# Autodesk Inventor assembly: Ensamblaje
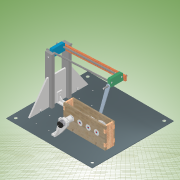
[picture p0: Inventor's stored thumbnail of the model, 180x180]
Saved by Autodesk Inventor 2022 (Build 260153000, 153)
## iProperties
Created: 2022-02-04
Part Number: Ensamblaje
Document SubType Name: Assembly
Designer: Marco
Author: Marco
## Documents named in this file (24)
- C:\Users\steff\Desktop\9noSemestre\Diseño\MiniProyecto\Ensamblaje.iam
- C:\Users\steff\Desktop\9noSemestre\Diseño\MiniProyecto\SoporteDerecha.ipt
- C:\Users\steff\Desktop\9noSemestre\Diseño\MiniProyecto\Varilla.ipt
- C:\Users\steff\Desktop\9noSemestre\Diseño\MiniProyecto\Riel_Lateral_MDF.ipt
- C:\Users\steff\Desktop\9noSemestre\Diseño\MiniProyecto\ColumnaSoporte.ipt
- C:\Users\steff\Desktop\9noSemestre\Diseño\MiniProyecto\SoporteIzquierda.ipt
- C:\Users\steff\Desktop\9noSemestre\Diseño\MiniProyecto\UnionColumnas.ipt
- C:\Users\steff\Desktop\9noSemestre\Diseño\MiniProyecto\SoporteMotor.ipt
- C:\Users\steff\Desktop\9noSemestre\Diseño\MiniProyecto\BaseProyecto.ipt
- C:\Users\steff\Desktop\9noSemestre\Diseño\MiniProyecto\CaraLateral.ipt
- C:\Users\steff\Desktop\9noSemestre\Diseño\MiniProyecto\Caja_CaraFrontal.ipt
- C:\Users\steff\Desktop\9noSemestre\Diseño\MiniProyecto\Rodamiento.ipt
- C:\Users\steff\Desktop\9noSemestre\Diseño\MiniProyecto\AcopleRod.ipt
- C:\Users\steff\Desktop\9noSemestre\Diseño\MiniProyecto\Eje.ipt
- C:\Users\steff\Desktop\9noSemestre\Diseño\MiniProyecto\Piñon1.ipt
- C:\Users\steff\Desktop\9noSemestre\Diseño\MiniProyecto\Archivos STL\EngranajesPegados.iam
- C:\Users\steff\Desktop\9noSemestre\Diseño\MiniProyecto\Engranaje1.ipt
- C:\Users\steff\Desktop\9noSemestre\Diseño\MiniProyecto\Transmision_Inf.ipt
- C:\Users\steff\Desktop\9noSemestre\Diseño\MiniProyecto\Transmision_Sup.ipt
- C:\Users\steff\Desktop\9noSemestre\Diseño\MiniProyecto\VarillaLateral.ipt
- C:\Users\steff\Desktop\9noSemestre\Diseño\MiniProyecto\AcopleMotor.ipt
- C:\Users\steff\Desktop\9noSemestre\Diseño\MiniProyecto\MotorDC.ipt
- C:\Users\steff\Desktop\9noSemestre\Diseño\MiniProyecto\SoporteMotorCierre.ipt
- C:\Users\steff\Desktop\9noSemestre\Diseño\MiniProyecto\Escuadra.ipt
## Components (44 placed, 23 different names)
1. BaseProyecto:1 — Coincidencia:1, Coincidencia:2, Coincidencia:3, Coincidencia:4, Coincidencia:5, Coincidencia:6, Coincidencia:13, Coincidencia:14, Coincidencia:15, Coincidencia:32, Coincidencia:33, Coincidencia:59
2. CaraLateral:1 — Coincidencia:1, Coincidencia:2, Coincidencia:3, Coincidencia:7, Coincidencia:8, Coincidencia:9, Coincidencia:11, Coincidencia:12, Coincidencia:34, Coincidencia:35, Coincidencia:36, Coincidencia:37, Coincidencia:38, Coincidencia:39, Coincidencia:40, Coincidencia:41
3. CaraLateral:2 — Coincidencia:4, Coincidencia:5, Coincidencia:6, Coincidencia:10, Coincidencia:42, Coincidencia:43, Coincidencia:44, Coincidencia:45, Coincidencia:46, Coincidencia:47
4. Caja_CaraFrontal:1 — Coincidencia:10, Coincidencia:11, Coincidencia:12
5. Caja_CaraFrontal:2 — Coincidencia:7, Coincidencia:8, Coincidencia:9
6. ColumnaSoporte:1 — Coincidencia:16, Coincidencia:17, De rotación:1, Coincidencia:20, Coincidencia:21, Coincidencia:51, Coincidencia:52
7. ColumnaSoporte:2 — Coincidencia:18, Coincidencia:19, Coincidencia:22, Coincidencia:23
8. UnionColumnas:1 — Coincidencia:13, Coincidencia:14, Coincidencia:15, Coincidencia:16, Coincidencia:17, Coincidencia:18, Coincidencia:19, Coincidencia:21, Coincidencia:22, Coincidencia:58, Coincidencia:60
9. SoporteIzquierda:1 — De rotación:1, De rotación:2, Coincidencia:20, Coincidencia:24, Coincidencia:25
10. Riel_Lateral_MDF:1 — De rotación:2, Coincidencia:23, Coincidencia:26, Coincidencia:27, Coincidencia:53
11. SoporteDerecha:1 — Coincidencia:26, Coincidencia:27, Coincidencia:28, Coincidencia:29, Coincidencia:30, Coincidencia:31, Coincidencia:49
12. Varilla:1 — Coincidencia:25, Coincidencia:29, Coincidencia:30
13. Varilla:2 — Coincidencia:24, Coincidencia:28, Coincidencia:31
14. SoporteMotor:1 — Coincidencia:32, Coincidencia:33, Coincidencia:54, Coincidencia:55, Coincidencia:56, Coincidencia:57
15. Rodamiento:1 — Coincidencia:34, Coincidencia:38, De rotación:3
16. Rodamiento:2 — Coincidencia:35, Coincidencia:39, De rotación:4
17. Rodamiento:3 — Coincidencia:37, Coincidencia:41, De rotación:6
18. Rodamiento:4 — Coincidencia:36, Coincidencia:40, De rotación:5
19. Rodamiento:5 — Coincidencia:46, Coincidencia:47, De rotación:9
20. Rodamiento:6 — Coincidencia:44, Coincidencia:45, De rotación:8
21. Rodamiento:8 — Coincidencia:42, Coincidencia:43, De rotación:7, De rotación:10
22. AcopleRod:1 — De rotación:6, Rígido:4
23. AcopleRod:2 — De rotación:4, Rígido:3
24. AcopleRod:3 — De rotación:5, Rígido:1
25. AcopleRod:4 — De rotación:3, Rígido:2
26. AcopleRod:5 — De rotación:7
27. AcopleRod:6 — De rotación:9
28. AcopleRod:7 — De rotación:8
29. Eje:4 — Rígido:1, Rígido:8
30. Eje:5 — Rígido:2, Rígido:5, Rígido:9
31. Eje:6 — Rígido:3, Rígido:6
32. Eje:7 — Rígido:4, Rígido:7
33. Piñon1:1 — Rígido:5
34. EngranajesPegados:1 [sub-assembly] — Rígido:8
35. EngranajesPegados:2 [sub-assembly] — Rígido:6
36. Engranaje1:1 — Rígido:7
37. Transmision_Inf:1 — De rotación:10, Coincidencia:48, De rotación:11
38. Transmision_Sup:1 — Coincidencia:48, De rotación:11, Coincidencia:49, Coincidencia:50
39. VarillaLateral:1 — Coincidencia:51, Coincidencia:52
40. VarillaLateral:2 — Coincidencia:50, Coincidencia:53
41. AcopleMotor:1 — Rígido:9
42. MotorDC:1 — Coincidencia:54, Coincidencia:55
43. SoporteMotorCierre:1 — Coincidencia:56, Coincidencia:57
44. Escuadra:1 — Coincidencia:58, Coincidencia:59, Coincidencia:60
## Relationships (80: Mate 60, RevoluteJoint 11, WeldJoint 9)
- Coincidencia:1 [Mate]: BaseProyecto:1 ↔ CaraLateral:1
- Coincidencia:2 [Mate]: BaseProyecto:1 ↔ CaraLateral:1
- Coincidencia:3 [Mate]: BaseProyecto:1 ↔ CaraLateral:1
- Coincidencia:4 [Mate]: BaseProyecto:1 ↔ CaraLateral:2
- Coincidencia:5 [Mate]: BaseProyecto:1 ↔ CaraLateral:2
- Coincidencia:6 [Mate]: BaseProyecto:1 ↔ CaraLateral:2
- Coincidencia:7 [Mate]: CaraLateral:1 ↔ Caja_CaraFrontal:2
- Coincidencia:8 [Mate]: CaraLateral:1 ↔ Caja_CaraFrontal:2
- Coincidencia:9 [Mate]: CaraLateral:1 ↔ Caja_CaraFrontal:2
- Coincidencia:10 [Mate]: CaraLateral:2 ↔ Caja_CaraFrontal:1
- Coincidencia:11 [Mate]: CaraLateral:1 ↔ Caja_CaraFrontal:1
- Coincidencia:12 [Mate]: CaraLateral:1 ↔ Caja_CaraFrontal:1
- Coincidencia:13 [Mate]: BaseProyecto:1 ↔ UnionColumnas:1
- Coincidencia:14 [Mate]: BaseProyecto:1 ↔ UnionColumnas:1
- Coincidencia:15 [Mate]: BaseProyecto:1 ↔ UnionColumnas:1
- Coincidencia:16 [Mate]: ColumnaSoporte:1 ↔ UnionColumnas:1
- Coincidencia:17 [Mate]: ColumnaSoporte:1 ↔ UnionColumnas:1
- Coincidencia:18 [Mate]: ColumnaSoporte:2 ↔ UnionColumnas:1
- Coincidencia:19 [Mate]: ColumnaSoporte:2 ↔ UnionColumnas:1
- De rotación:1 [RevoluteJoint]: ColumnaSoporte:1 ↔ SoporteIzquierda:1
- De rotación:2 [RevoluteJoint]: SoporteIzquierda:1 ↔ Riel_Lateral_MDF:1
- Coincidencia:20 [Mate]: ColumnaSoporte:1 ↔ SoporteIzquierda:1
- Coincidencia:21 [Mate]: ColumnaSoporte:1 ↔ UnionColumnas:1
- Coincidencia:22 [Mate]: ColumnaSoporte:2 ↔ UnionColumnas:1
- Coincidencia:23 [Mate]: ColumnaSoporte:2 ↔ Riel_Lateral_MDF:1
- Coincidencia:24 [Mate]: SoporteIzquierda:1 ↔ Varilla:2
- Coincidencia:25 [Mate]: SoporteIzquierda:1 ↔ Varilla:1
- Coincidencia:26 [Mate]: Riel_Lateral_MDF:1 ↔ SoporteDerecha:1
- Coincidencia:27 [Mate]: Riel_Lateral_MDF:1 ↔ SoporteDerecha:1
- Coincidencia:28 [Mate]: SoporteDerecha:1 ↔ Varilla:2
- Coincidencia:29 [Mate]: SoporteDerecha:1 ↔ Varilla:1
- Coincidencia:30 [Mate]: SoporteDerecha:1 ↔ Varilla:1
- Coincidencia:31 [Mate]: SoporteDerecha:1 ↔ Varilla:2
- Coincidencia:32 [Mate]: BaseProyecto:1 ↔ SoporteMotor:1
- Coincidencia:33 [Mate]: BaseProyecto:1 ↔ SoporteMotor:1
- Coincidencia:34 [Mate]: CaraLateral:1 ↔ Rodamiento:1
- Coincidencia:35 [Mate]: CaraLateral:1 ↔ Rodamiento:2
- Coincidencia:36 [Mate]: CaraLateral:1 ↔ Rodamiento:4
- Coincidencia:37 [Mate]: CaraLateral:1 ↔ Rodamiento:3
- Coincidencia:38 [Mate]: CaraLateral:1 ↔ Rodamiento:1
- Coincidencia:39 [Mate]: CaraLateral:1 ↔ Rodamiento:2
- Coincidencia:40 [Mate]: CaraLateral:1 ↔ Rodamiento:4
- Coincidencia:41 [Mate]: CaraLateral:1 ↔ Rodamiento:3
- Coincidencia:42 [Mate]: CaraLateral:2 ↔ Rodamiento:8
- Coincidencia:43 [Mate]: CaraLateral:2 ↔ Rodamiento:8
- Coincidencia:44 [Mate]: CaraLateral:2 ↔ Rodamiento:6
- Coincidencia:45 [Mate]: CaraLateral:2 ↔ Rodamiento:6
- Coincidencia:46 [Mate]: CaraLateral:2 ↔ Rodamiento:5
- Coincidencia:47 [Mate]: CaraLateral:2 ↔ Rodamiento:5
- De rotación:3 [RevoluteJoint]: Rodamiento:1 ↔ AcopleRod:4
- De rotación:4 [RevoluteJoint]: Rodamiento:2 ↔ AcopleRod:2
- De rotación:5 [RevoluteJoint]: Rodamiento:4 ↔ AcopleRod:3
- De rotación:6 [RevoluteJoint]: Rodamiento:3 ↔ AcopleRod:1
- De rotación:7 [RevoluteJoint]: Rodamiento:8 ↔ AcopleRod:5
- De rotación:8 [RevoluteJoint]: Rodamiento:6 ↔ AcopleRod:7
- De rotación:9 [RevoluteJoint]: Rodamiento:5 ↔ AcopleRod:6
- Rígido:1 [WeldJoint]: AcopleRod:3 ↔ Eje:4
- Rígido:2 [WeldJoint] (-40 mm): AcopleRod:4 ↔ Eje:5
- Rígido:3 [WeldJoint] (-45 mm): AcopleRod:2 ↔ Eje:6
- Rígido:4 [WeldJoint] (-45 mm): AcopleRod:1 ↔ Eje:7
- Rígido:5 [WeldJoint] (-18 mm): Eje:5 ↔ Piñon1:1
- Rígido:6 [WeldJoint] (-20 mm): Eje:6 ↔ EngranajesPegados:2
- Rígido:7 [WeldJoint] (-28 mm): Eje:7 ↔ Engranaje1:1
- Rígido:8 [WeldJoint] (-27 mm): Eje:4 ↔ EngranajesPegados:1
- De rotación:10 [RevoluteJoint]: Rodamiento:8 ↔ Transmision_Inf:1
- Coincidencia:48 [Mate]: Transmision_Inf:1 ↔ Transmision_Sup:1
- De rotación:11 [RevoluteJoint]: Transmision_Inf:1 ↔ Transmision_Sup:1
- Coincidencia:49 [Mate]: SoporteDerecha:1 ↔ Transmision_Sup:1
- Coincidencia:50 [Mate]: Transmision_Sup:1 ↔ VarillaLateral:2
- Coincidencia:51 [Mate]: ColumnaSoporte:1 ↔ VarillaLateral:1
- Coincidencia:52 [Mate]: ColumnaSoporte:1 ↔ VarillaLateral:1
- Coincidencia:53 [Mate] (15 mm): Riel_Lateral_MDF:1 ↔ VarillaLateral:2
- Rígido:9 [WeldJoint]: Eje:5 ↔ AcopleMotor:1
- Coincidencia:54 [Mate]: SoporteMotor:1 ↔ MotorDC:1
- Coincidencia:55 [Mate]: SoporteMotor:1 ↔ MotorDC:1
- Coincidencia:56 [Mate]: SoporteMotor:1 ↔ SoporteMotorCierre:1
- Coincidencia:57 [Mate]: SoporteMotor:1 ↔ SoporteMotorCierre:1
- Coincidencia:58 [Mate]: UnionColumnas:1 ↔ Escuadra:1
- Coincidencia:59 [Mate]: BaseProyecto:1 ↔ Escuadra:1
- Coincidencia:60 [Mate]: UnionColumnas:1 ↔ Escuadra:1
